# Autodesk Inventor assembly: ASY GNH 011 Dilution point Frame1
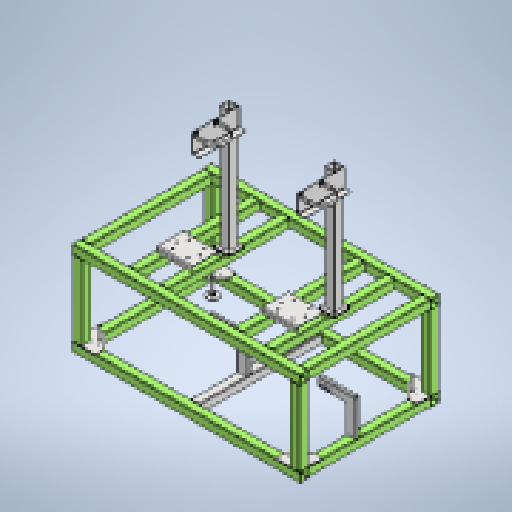
[picture p0: Inventor's stored thumbnail of the model, 512x512]
Saved by Autodesk Inventor 2025.1 (Build 291241020, 241B)
## iProperties
Created: 2025-03-06
Part Number: ASY GNH 011 Dilution point Frame1
Document SubType Name: Assembly
Designer: user
_SolveAssemblyDoc: Frame Generator Solve Assembly
_Version: 25.0.0
Author: user
## Documents named in this file (11)
- C:\Users\user\YandexDisk-badmisterfox\home pc\Inventor\GNH-Petrodvorec\ASY GNH 011 Dilution point Frame1.iam
- C:\Users\user\YandexDisk-badmisterfox\home pc\Inventor\GNH-Petrodvorec\GNH 011 Dilution frame sketch.ipt
- C:\Users\user\YandexDisk-badmisterfox\home pc\Inventor\GNH-Petrodvorec\ASY GNH 010 Dilution point Frame\Frame\Frame 1741245058463.iam
- C:\Users\user\YandexDisk-badmisterfox\home pc\Inventor\GNH-Petrodvorec\GNH 015 leg support.ipt
- C:\Users\user\YandexDisk-badmisterfox\home pc\Inventor\GNH-Petrodvorec\Content Center Files\en-US\ISO 8676(1)\ISO 8676 - M12 x 1.25 x 120DIN EN.ipt
- C:\Users\user\YandexDisk-badmisterfox\home pc\Inventor\GNH-Petrodvorec\GNH 015 leg plate.ipt
- C:\Users\user\YandexDisk-badmisterfox\home pc\Inventor\GNH-Petrodvorec\GNH 016  Motor pillar.ipt
- C:\Users\user\YandexDisk-badmisterfox\home pc\Inventor\GNH-Petrodvorec\GNH 017  Pulse compensator.ipt
- C:\Users\user\YandexDisk-badmisterfox\home pc\Inventor\GNH-Petrodvorec\GNH 018  Plate pulse pillar.ipt
- C:\Users\user\YandexDisk-badmisterfox\home pc\Inventor\GNH-Petrodvorec\GNH 019  Valve pillar.ipt
- C:\Users\user\YandexDisk-badmisterfox\home pc\Inventor\GNH-Petrodvorec\stainer Cradle 4.ipt
## Components (26 placed, 12 different names)
1. GNH 011 Dilution frame sketch:1
2. Frame 1741245058463:1 [sub-assembly] — Mate:1, Flush:1, Flush:2, Rigid:3, Rigid:4, Rigid:5, Mate:2, Flush:3, Flush:4, Rigid:14, Rigid:15, Rigid:17, Rigid:19, Rigid:20, Rigid:21
3. GNH 081 leg support:1 — Mate:1, Flush:1, Flush:2, Rigid:9
4. ISO 8676 - M12 x 1.25 x 120:1 — Rigid:2, Rigid:9
5. GNH 082 leg plate:1 — Rigid:2
6. MNT-CDF-604 CAP:4 — Rigid:4, Rigid:12
7. MNT-CDF-604 CAP:5 — Rigid:3, Rigid:10
8. MNT-CDF-604 CAP:6 — Rigid:5, Rigid:11
9. DIN EN 28676 M12 x 1.25 x 120:2 — Rigid:8, Rigid:10
10. DIN EN 28676 M12 x 1.25 x 120:3 — Rigid:7, Rigid:12
11. DIN EN 28676 M12 x 1.25 x 120:4 — Rigid:6, Rigid:11
12. MNT-CDF-604 CAP:7 — Rigid:8
13. MNT-CDF-604 CAP:8 — Rigid:7
14. MNT-CDF-604 CAP:9 — Rigid:6
15. GNH 016  Motor pillar:1 — Mate:2, Flush:3, Flush:4, Rigid:13
16. GNH 016  Motor pillar:2 — Rigid:13
17. GNH 017  Pulse compensator:1 — Rigid:14, Rigid:22
18. GNH 017  Pulse compensator:2 — Rigid:15, Rigid:23
19. GNH 018  Plate pulse pillar:1 — Rigid:16, Rigid:17
20. GNH 018  Plate pulse pillar:2 — Rigid:16
21. GNH 018  Plate pulse pillar:3 — Rigid:19
22. GNH 018  Plate pulse pillar:4
23. GNH 019  Valve pillar:1 — Rigid:20
24. GNH 019  Valve pillar:2 — Rigid:21
25. stainer Cradle 4:1 — Rigid:22
26. stainer Cradle 4:2 — Rigid:23
## Relationships (28: WeldJoint 22, Flush 4, Mate 2)
- Mate:1: Frame 1741245058463:1 ↔ GNH 081 leg support:1
- Flush:1: Frame 1741245058463:1 ↔ GNH 081 leg support:1
- Flush:2: Frame 1741245058463:1 ↔ GNH 081 leg support:1
- Rigid:2 [WeldJoint]: ISO 8676 - M12 x 1.25 x 120:1 ↔ GNH 082 leg plate:1
- Rigid:3 [WeldJoint]: Frame 1741245058463:1 ↔ MNT-CDF-604 CAP:5
- Rigid:4 [WeldJoint]: Frame 1741245058463:1 ↔ MNT-CDF-604 CAP:4
- Rigid:5 [WeldJoint]: Frame 1741245058463:1 ↔ MNT-CDF-604 CAP:6
- Rigid:6 [WeldJoint]: DIN EN 28676 M12 x 1.25 x 120:4 ↔ MNT-CDF-604 CAP:9
- Rigid:7 [WeldJoint]: DIN EN 28676 M12 x 1.25 x 120:3 ↔ MNT-CDF-604 CAP:8
- Rigid:8 [WeldJoint]: DIN EN 28676 M12 x 1.25 x 120:2 ↔ MNT-CDF-604 CAP:7
- Rigid:9 [WeldJoint]: GNH 081 leg support:1 ↔ ISO 8676 - M12 x 1.25 x 120:1
- Rigid:10 [WeldJoint]: MNT-CDF-604 CAP:5 ↔ DIN EN 28676 M12 x 1.25 x 120:2
- Rigid:11 [WeldJoint]: MNT-CDF-604 CAP:6 ↔ DIN EN 28676 M12 x 1.25 x 120:4
- Rigid:12 [WeldJoint]: MNT-CDF-604 CAP:4 ↔ DIN EN 28676 M12 x 1.25 x 120:3
- Mate:2: Frame 1741245058463:1 ↔ GNH 016  Motor pillar:1
- Flush:3 (10 mm): Frame 1741245058463:1 ↔ GNH 016  Motor pillar:1
- Flush:4 (150 mm): Frame 1741245058463:1 ↔ GNH 016  Motor pillar:1
- Rigid:13 [WeldJoint] (-450 mm): GNH 016  Motor pillar:1 ↔ GNH 016  Motor pillar:2
- Rigid:14 [WeldJoint]: Frame 1741245058463:1 ↔ GNH 017  Pulse compensator:1
- Rigid:15 [WeldJoint]: Frame 1741245058463:1 ↔ GNH 017  Pulse compensator:2
- Rigid:16 [WeldJoint]: GNH 018  Plate pulse pillar:1 ↔ GNH 018  Plate pulse pillar:2
- Rigid:17 [WeldJoint]: Frame 1741245058463:1 ↔ GNH 018  Plate pulse pillar:1
- [WeldJoint]: GNH 018  Plate pulse pillar:3 ↔ GNH 018  Plate pulse pillar:4
- Rigid:19 [WeldJoint]: Frame 1741245058463:1 ↔ GNH 018  Plate pulse pillar:3
- Rigid:20 [WeldJoint] (200 mm): Frame 1741245058463:1 ↔ GNH 019  Valve pillar:1
- Rigid:21 [WeldJoint] (-200 mm): Frame 1741245058463:1 ↔ GNH 019  Valve pillar:2
- Rigid:22 [WeldJoint] (-5 mm): GNH 017  Pulse compensator:1 ↔ stainer Cradle 4:1
- Rigid:23 [WeldJoint] (-5 mm): GNH 017  Pulse compensator:2 ↔ stainer Cradle 4:2
## Named parameters: d29_d27 = 0 mm
